# Autodesk Inventor assembly: twopart_track_assembly
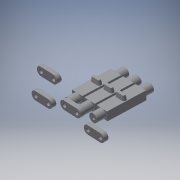
[picture p0: Inventor's stored thumbnail of the model, 180x180]
Saved by Autodesk Inventor 2016 (Build 200138000, 138)
## iProperties
Created: 2016-05-02
Part Number: twopart_track_assembly
Document SubType Name: Assembly
Designer: Henrik Samuelsson
Author: Henrik Samuelsson
## Documents named in this file (3)
- C:\Users\Henrik Samuelsson\Documents\Killer-Bot-2016\AutodeskWorkspace\twopart_track_assembly.iam
- C:\Users\Henrik Samuelsson\Documents\Killer-Bot-2016\AutodeskWorkspace\tracks_center.ipt
- C:\Users\Henrik Samuelsson\Documents\Killer-Bot-2016\AutodeskWorkspace\tracks_outer.ipt
## Components (7 placed, 2 different names)
1. tracks_center:1 — Flush:1, Insert:4
2. tracks_center:2 — Insert:1, Insert:2, Flush:1
3. tracks_center:3 — Insert:3
4. tracks_outer:1 — Flush:3
5. tracks_outer:2 — Flush:4
6. tracks_outer:3 — Insert:1, Insert:2, Flush:2, Flush:4, Insert:3, Insert:4
7. tracks_outer:4 — Flush:2, Flush:3
## Relationships (8: Insert 4, Flush 4)
- Insert:1: tracks_center:2 ↔ tracks_outer:3
- Insert:2: tracks_center:2 ↔ tracks_outer:3
- Flush:1: tracks_center:1 ↔ tracks_center:2
- Flush:2: tracks_outer:3 ↔ tracks_outer:4
- Flush:3: tracks_outer:1 ↔ tracks_outer:4
- Flush:4: tracks_outer:2 ↔ tracks_outer:3
- Insert:3: tracks_center:3 ↔ tracks_outer:3
- Insert:4: tracks_center:1 ↔ tracks_outer:3
